# Autodesk Inventor assembly: EBF_910.1-eb-flow
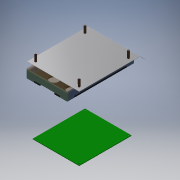
[picture p0: Inventor's stored thumbnail of the model, 180x180]
Saved by Autodesk Inventor 2019 (Build 230136000, 136)
## iProperties
Created: 2019-03-05
Part Number: EBF_910.1-eb-flow
Document SubType Name: Assembly
Designer: Rene
Author: Rene
## Documents named in this file (4)
- C:\dev\c-scape\hardponics\dwg\eb_flow\EBF_910.1-eb-flow.iam
- C:\dev\c-scape\hardponics\dwg\eb_flow\XGEN_hotbed-pcb.ipt
- C:\dev\c-scape\hardponics\dwg\eb_flow\EBF_900.1-water-tray_with_cups.iam
- C:\dev\c-scape\hardponics\dwg\eb_flow\XGEN_simsun-pcb.ipt
## Components (3 placed, 3 different names)
1. XGEN_hotbed-pcb:1 — Mate:1, Mate:2, Mate:3, Mate:4, Mate:5
2. EBF_900.1-water-tray_with_cups:1 [sub-assembly] — Mate:1, Mate:2
3. XGEN_simsun-pcb:1 — Mate:3, Mate:4, Mate:5
## Relationships (5: Mate 5)
- Mate:1: XGEN_hotbed-pcb:1 ↔ EBF_900.1-water-tray_with_cups:1
- Mate:2: XGEN_hotbed-pcb:1 ↔ EBF_900.1-water-tray_with_cups:1
- Mate:3: XGEN_hotbed-pcb:1 ↔ XGEN_simsun-pcb:1
- Mate:4: XGEN_hotbed-pcb:1 ↔ XGEN_simsun-pcb:1
- Mate:5 (230 mm): XGEN_hotbed-pcb:1 ↔ XGEN_simsun-pcb:1
